# Autodesk Inventor assembly: flame_side_right
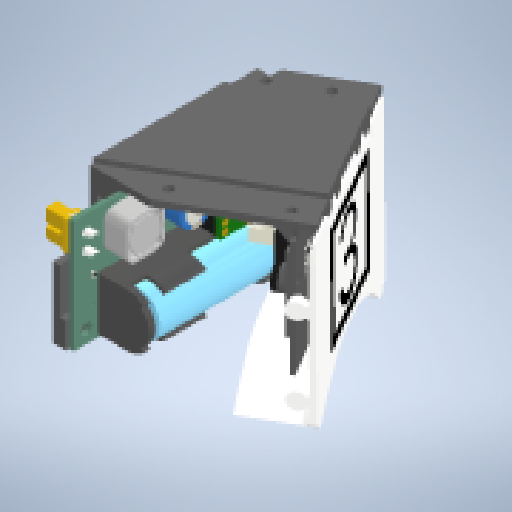
[picture p0: Inventor's stored thumbnail of the model, 512x512]
Saved by Autodesk Inventor 2024.1 (Build 281209000, 209)
## iProperties
Created: 2025-04-22
Part Number: flame_side_right
Document SubType Name: Assembly
Designer: hibik
Author: hibik
## Documents named in this file (5)
- C:\Users\hibik\Documents\Robomech\RESCUE\ORCA\hard\flame_back\Assy_flame_side_right.iam
- C:\Users\hibik\Documents\Robomech\RESCUE\ORCA\hard\flame_back\flame_side_right.ipt
- C:\Users\hibik\Documents\Robomech\RESCUE\ORCA\hard\board\power_model\usp.iam
- C:\Users\hibik\Documents\Robomech\RESCUE\ORCA\hard\cover\cover_side.ipt
- C:\Users\hibik\Documents\Robomech\RESCUE\ORCA\hard\board\CORE_model\external_io_reset.iam
## Components (4 placed, 4 different names)
1. flame_side_right:1 — 挿入:1, 角度:1, 挿入:2, 角度:2, 挿入:3
2. usp:1 [sub-assembly] — 挿入:1, 角度:1
3. cover_side:1 — 挿入:2
4. external_io_reset:1 [sub-assembly] — 角度:2, 挿入:3
## Relationships (5: Insert 3, Angle 2)
- 挿入:1 [Insert]: flame_side_right:1 ↔ usp:1
- 角度:1 [Angle] (0 deg): flame_side_right:1 ↔ usp:1
- 挿入:2 [Insert] (0.25 mm): flame_side_right:1 ↔ cover_side:1
- 角度:2 [Angle] (0 deg): flame_side_right:1 ↔ external_io_reset:1
- 挿入:3 [Insert]: flame_side_right:1 ↔ external_io_reset:1
